# Autodesk Inventor assembly: Rack and Pinion Gear
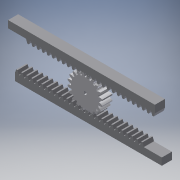
[picture p0: Inventor's stored thumbnail of the model, 180x180]
Saved by Autodesk Inventor 2016 (Build 200138000, 138)
## iProperties
Created: 2016-04-02
Part Number: Rack and Pinion Gear
Document SubType Name: Assembly
Designer: amycroft3
Author: amycroft3
## Documents named in this file (4)
- C:\Users\Andrea\Documents\Dropbox\Capstone CAD\Rack and Pinion Gear.iam
- C:\Users\Andrea\Documents\Dropbox\Capstone CAD\Pinion Gear.ipt
- C:\Users\Andrea\Documents\Dropbox\Capstone CAD\Upper Rack.ipt
- C:\Users\Andrea\Documents\Dropbox\Capstone CAD\Lower Rack.ipt
## Components (3 placed, 3 different names)
1. Pinion Gear:1 — Mate:1, Mate:2, Flush:1, Tangent:2, Rotation/Translation:2, Tangent:3, Rotation/Translation:3, Mate:3
2. Lower Rack:1 — Angle:1, Angle:2, Tangent:3, Angle:3, Rotation/Translation:3, Mate:3, Mate:5
3. Upper Rack:1 — Flush:1, Tangent:2, Rotation/Translation:2, Angle:2, Angle:3, Mate:4, Mate:5
## Relationships (13: Mate 5, Angle 3, Tangent 2, RelateRotateTranslate 2, Flush 1)
- Mate:1: Pinion Gear:1
- Mate:2: Pinion Gear:1
- Angle:1 (0 deg): Lower Rack:1
- Flush:1: Pinion Gear:1 ↔ Upper Rack:1
- Tangent:2: Pinion Gear:1 ↔ Upper Rack:1
- Rotation/Translation:2 [RelateRotateTranslate] (50.8 mm): Pinion Gear:1 ↔ Upper Rack:1
- Angle:2 (180 deg): Lower Rack:1 ↔ Upper Rack:1
- Tangent:3: Pinion Gear:1 ↔ Lower Rack:1
- Angle:3 (0 deg): Lower Rack:1 ↔ Upper Rack:1
- Rotation/Translation:3 [RelateRotateTranslate] (50.8 mm): Pinion Gear:1 ↔ Lower Rack:1
- Mate:3: Pinion Gear:1 ↔ Lower Rack:1
- Mate:4: Upper Rack:1
- Mate:5: Lower Rack:1 ↔ Upper Rack:1
